# Autodesk Inventor assembly: Grundplatte_ZSB
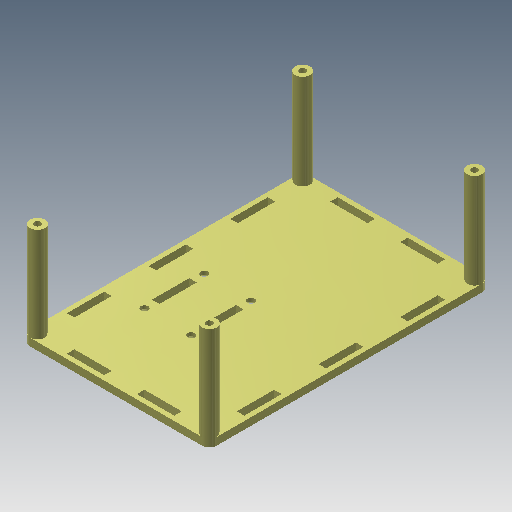
[picture p0: Inventor's stored thumbnail of the model, 512x512]
Saved by Autodesk Inventor 2019 (Build 230136000, 136)
## iProperties
Created: 2022-11-01
Part Number: Grundplatte_ZSB
Material: Generisch
Document SubType Name: Assembly
Designer: RP
Author: RP
## Documents named in this file (5)
- C:\Users\RP\Documents\Inventor\___Projekt_Useless_Box\_Useless_Box\Grundplatte_ZSB.iam
- C:\Users\RP\Documents\Inventor\___Projekt_Useless_Box\_Useless_Box\Grundplatte.ipt
- C:\Users\RP\Documents\Inventor\___Projekt_Useless_Box\_Useless_Box\Side dowel UM_D‚faut.ipt
- C:\Users\RP\Documents\Inventor\___Projekt_Useless_Box\_Useless_Box\Gewinderohr.ipt
- C:\Users\RP\Documents\Inventor\___Projekt_Useless_Box\_Useless_Box\ISO 10642  - M4  x  16.ipt
## Components (9 placed, 3 different names)
1. Grundplatte:1 — Fluchtend:1, Fluchtend:2, Fluchtend:3
2. Gewinderohr:1
3. Gewinderohr:2
4. Gewinderohr:3
5. Gewinderohr:4
6. DIN EN ISO 10642 M4  x  16:1
7. DIN EN ISO 10642 M4  x  16:2
8. DIN EN ISO 10642 M4  x  16:3
9. DIN EN ISO 10642 M4  x  16:4
## Relationships (11: Insert 8, Flush 3)
- [Insert]: Grundplatte:1 ↔ Gewinderohr:2
- [Insert]: Grundplatte:1 ↔ Gewinderohr:1
- [Insert]: Grundplatte:1 ↔ Gewinderohr:4
- [Insert]: Grundplatte:1 ↔ Gewinderohr:3
- [Insert]: Grundplatte:1 ↔ DIN EN ISO 10642 M4  x  16:1
- [Insert]: Grundplatte:1 ↔ DIN EN ISO 10642 M4  x  16:2
- [Insert]: Grundplatte:1 ↔ DIN EN ISO 10642 M4  x  16:4
- [Insert]: Grundplatte:1 ↔ DIN EN ISO 10642 M4  x  16:3
- Fluchtend:1 [Flush] (-50 mm): Grundplatte:1
- Fluchtend:2 [Flush] (-70 mm): Grundplatte:1
- Fluchtend:3 [Flush]: Grundplatte:1
